# Autodesk Inventor assembly: Ensamblaje3
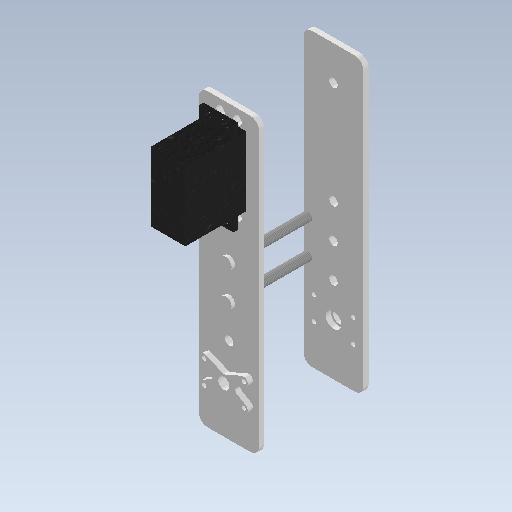
[picture p0: Inventor's stored thumbnail of the model, 512x512]
Saved by Autodesk Inventor 2021 (Build 250183000, 183)
## iProperties
Created: 2021-04-03
Part Number: Ensamblaje3
Document SubType Name: Assembly
Designer: diego
Author: diego
## Documents named in this file (6)
- C:\Users\diego\Desktop\Diego\Utadeo 2021-1\Robotica Industrial\Corte 2\Solido planos\Ensamblaje3.iam
- C:\Users\diego\Desktop\Diego\Utadeo 2021-1\Robotica Industrial\Corte 2\Solido planos\1.ipt
- C:\Users\diego\Desktop\Diego\Utadeo 2021-1\Robotica Industrial\Corte 2\Solido planos\Extension2.ipt
- C:\Users\diego\Desktop\Diego\Utadeo 2021-1\Robotica Industrial\Corte 2\Solido planos\Tornillo_Corto.ipt
- C:\Users\diego\Desktop\Diego\Utadeo 2021-1\Robotica Industrial\Corte 2\Solido planos\Servo.ipt
- C:\Users\diego\Desktop\Diego\Utadeo 2021-1\Robotica Industrial\Corte 2\Solido planos\2.ipt
## Components (7 placed, 5 different names)
1. 1:1 — Coincidencia:1, Coincidencia:2, De rotación:1, Rígido:1, Rígido:2
2. Extension2:1 — Coincidencia:1, Coincidencia:2
3. Servo:1 — De rotación:1
4. 2:1 — Coincidencia:3, Coincidencia:4, Rígido:3
5. Extension2:2 — Coincidencia:3, Coincidencia:4
6. Tornillo_Corto:1 — Rígido:2
7. Tornillo_Corto:2 — Rígido:1, Rígido:3
## Relationships (8: Mate 4, WeldJoint 3, RevoluteJoint 1)
- Coincidencia:1 [Mate]: 1:1 ↔ Extension2:1
- Coincidencia:2 [Mate]: 1:1 ↔ Extension2:1
- De rotación:1 [RevoluteJoint] (3 mm): 1:1 ↔ Servo:1
- Coincidencia:3 [Mate]: 2:1 ↔ Extension2:2
- Coincidencia:4 [Mate]: 2:1 ↔ Extension2:2
- Rígido:1 [WeldJoint]: 1:1 ↔ Tornillo_Corto:2
- Rígido:2 [WeldJoint]: 1:1 ↔ Tornillo_Corto:1
- Rígido:3 [WeldJoint] (-9 mm): 2:1 ↔ Tornillo_Corto:2
